# Autodesk Inventor assembly: subgpu
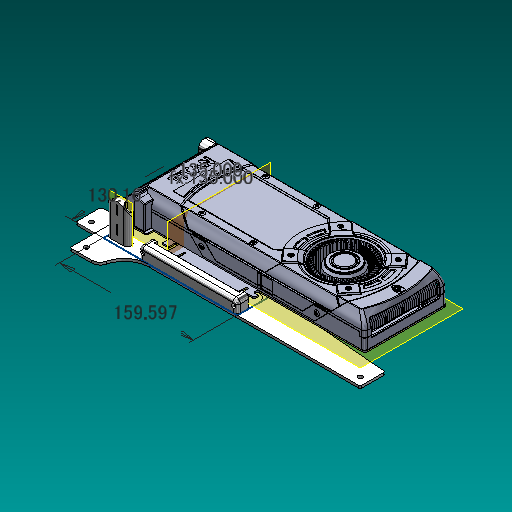
[picture p0: Inventor's stored thumbnail of the model, 512x512]
Saved by Autodesk Inventor 2018.2 (Build 222227000, 227)
## iProperties
Created: 2020-06-13
Part Number: subgpu
Material: 一般
Document SubType Name: Assembly
Designer: gisen
Author: gisen
## Documents named in this file (7)
- C:\Users\gisen\Documents\CAD\github\eatx_case\eatx_full\subgpu\subgpu.iam
- C:\Users\gisen\Documents\CAD\github\eatx_case\eatx_full\resources\gpu\titan assembly.iam
- C:\Users\gisen\Documents\CAD\github\eatx_case\eatx_full\parts\small_gpu_01.ipt
- C:\Users\gisen\Documents\CAD\github\eatx_case\eatx_full\parts\small_gpu_02.ipt
- C:\Users\gisen\Documents\CAD\github\eatx_case\eatx_full\parts\small_gpu_03.ipt
- C:\Users\gisen\Documents\CAD\github\eatx_case\eatx_full\parts\small_gpu_04.ipt
- C:\Users\gisen\Documents\CAD\github\eatx_case\eatx_full\parts\small_gpu_05.ipt
## Components (6 placed, 6 different names)
1. titan assembly:1 [sub-assembly] — メイト:1, メイト:2, 角度:1, メイト:3, メイト:4, フラッシュ:1, メイト:5, 角度:2, メイト:6, フラッシュ:2
2. small_gpu_01:1 — メイト:3, メイト:4, フラッシュ:1
3. small_gpu_02:1 — メイト:1, メイト:2, 角度:1
4. small_gpu_03:1 — メイト:5, 角度:2, メイト:6, フラッシュ:2, メイト:7, メイト:8, メイト:9, メイト:10, メイト:11, メイト:12
5. small_gpu_04:1 — メイト:7, メイト:8, メイト:9
6. small_gpu_05:1 — メイト:10, メイト:11, メイト:12
## Relationships (16: Mate 12, Angle 2, Flush 2)
- メイト:1 [Mate]: titan assembly:1 ↔ small_gpu_02:1
- メイト:2 [Mate]: titan assembly:1 ↔ small_gpu_02:1
- 角度:1 [Angle] (0 deg): titan assembly:1 ↔ small_gpu_02:1
- メイト:3 [Mate] (0.125 mm): titan assembly:1 ↔ small_gpu_01:1
- メイト:4 [Mate] (0.125 mm): titan assembly:1 ↔ small_gpu_01:1
- フラッシュ:1 [Flush]: titan assembly:1 ↔ small_gpu_01:1
- メイト:5 [Mate] (18.1 mm): titan assembly:1 ↔ small_gpu_03:1
- 角度:2 [Angle] (0 deg): titan assembly:1 ↔ small_gpu_03:1
- メイト:6 [Mate]: titan assembly:1 ↔ small_gpu_03:1
- フラッシュ:2 [Flush] (-4.6 mm): titan assembly:1 ↔ small_gpu_03:1
- メイト:7 [Mate]: small_gpu_03:1 ↔ small_gpu_04:1
- メイト:8 [Mate]: small_gpu_03:1 ↔ small_gpu_04:1
- メイト:9 [Mate]: small_gpu_03:1 ↔ small_gpu_04:1
- メイト:10 [Mate]: small_gpu_03:1 ↔ small_gpu_05:1
- メイト:11 [Mate]: small_gpu_03:1 ↔ small_gpu_05:1
- メイト:12 [Mate]: small_gpu_03:1 ↔ small_gpu_05:1
